# Autodesk Inventor assembly: plate attachment _MIR
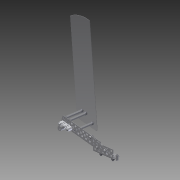
[picture p0: Inventor's stored thumbnail of the model, 180x180]
Saved by Autodesk Inventor 2014 SP1 (Build 180222100, 222)
## iProperties
Created: 2014-03-20
Part Number: plate attachment _MIR
Document SubType Name: Assembly
Designer: Ryan
Author: Ryan
## Documents named in this file (15)
- C:\Users\Ryan\Desktop\sw\toss up 5th A bot\intake\plate attachment _MIR.iam
- C:\Users\Ryan\Desktop\sw\lib\Aperture VEX CAD Library\Metal\L Bar\2 x 5.ipt
- C:\Users\Ryan\Desktop\sw\lib\Aperture VEX CAD Library\Metal\L Bar\2 x 10.ipt
- C:\Users\Ryan\Desktop\sw\lib\Aperture VEX CAD Library\Hardware\8-32\8-32_.375.ipt
- C:\Users\Ryan\Desktop\sw\lib\Aperture VEX CAD Library\Hardware\8-32\8-32 nylock_MIR12.ipt
- C:\Users\Ryan\Desktop\sw\lib\Aperture VEX CAD Library\Metal\Custom 1 bar\5.ipt
- C:\Users\Ryan\Desktop\sw\lib\Aperture VEX CAD Library\Hardware\8-32\8-32 nylock.ipt
- C:\Users\Ryan\Desktop\sw\lib\Aperture VEX CAD Library\Bearing Blocks\Bearing Block.ipt
- C:\Users\Ryan\Desktop\sw\lib\Aperture VEX CAD Library\Hardware\8-32\8-32_.250.ipt
- C:\Users\Ryan\Desktop\sw\lib\Aperture VEX CAD Library\Standoffs\BEAM-0500.ipt
- C:\Users\Ryan\Desktop\sw\lib\Aperture VEX CAD Library\Standoffs\BEAM-2000.ipt
- C:\Users\Ryan\Desktop\sw\lib\Aperture VEX CAD Library\Hardware\8-32\8-23_.750.ipt
- C:\Users\Ryan\Desktop\sw\lib\Aperture VEX CAD Library\Spacers\SPACER-0500-0125.ipt
- C:\Users\Ryan\Desktop\sw\lib\Aperture VEX CAD Library\Spacers\SPACER-0500-0375.ipt
- C:\Users\Ryan\Desktop\sw\toss up 5th A bot\intake\large ball holder.ipt
## Components (36 placed, 14 different names)
1. 2 x 5:1 — Mate:31, Mate:30, Mate:29, Mate:28, Mate:36, Mate:38, Mate:37, Mate:44, Mate:66, Mate:65, Mate:64, Mate:67, Mate:70, Mate:69, Mate:68, Flush:1
2. 2 x 10:1 — Mate:31, Mate:33, Mate:32, Mate:35, Mate:46, Mate:45, Mate:51, Mate:86, Mate:62, Mate:59, Mate:60, Mate:92, Mate:91, Mate:83, Mate:90, Mate:97, Mate:96, Mate:95
3. 8-32_.375:1 — Mate:33, Mate:32, Mate:30, Mate:29, Mate:28, Mate:34
4. 8-32 nylock_MIR12:1 — Mate:35, Mate:34
5. 5:1 — Mate:36, Mate:43, Mate:42, Mate:41, Mate:49, Mate:48, Mate:47
6. 8-32_.375:2 — Mate:43, Mate:42, Mate:41, Mate:38, Mate:37, Mate:40
7. 8-32 nylock:1 — Mate:44, Mate:40
8. 8-32_.375:3 — Mate:49, Mate:48, Mate:47, Mate:46, Mate:45, Mate:50
9. 8-32 nylock:2 — Mate:51, Mate:50
10. Bearing Block:1 — Mate:86, Mate:62, Mate:59, Mate:58, Mate:57, Mate:56, Mate:87
11. Bearing Block:2 — Mate:60, Mate:58, Mate:57, Mate:56, Mate:88, Mate:103, Mate:102
12. 8-32_.250:1 — Mate:70, Mate:69, Mate:68, Mate:71
13. BEAM-0500:1 — Flush:1, Mate:71
14. BEAM-2000:2 — Mate:93, Mate:94, Mate:99, Mate:98
15. 8-32 nylock:6 — Mate:97, Mate:96, Mate:95, Mate:93, Mate:94
16. 8-32 nylock:7 — Mate:99, Mate:98, Mate:107, Mate:106, Mate:66
17. SPACER-0500-0125:1 — Mate:103, Mate:102, Mate:105, Mate:104
18. SPACER-0500-0375:1 — Mate:105, Mate:104
19. 8-32_.375:5 — Mate:107, Mate:106, Mate:69
20. large ball holder:1 — Mate:66, Mate:69, Mate:70
21. 8-32 nylock:3 — Mate:67, Mate:63
22. 8-32_.375:4 — Mate:66, Mate:65, Mate:64, Mate:63
23. 8-32 nylock:9
24. 8-32_.375:7
25. 8-23_.750:1 — Mate:89, Mate:88, Mate:87
26. 8-32 nylock:5 — Mate:90, Mate:89
27. 8-23_.750:2
28. 8-32 nylock:10
29. BEAM-2000:1 — Mate:85, Mate:84, Mate:101, Mate:100
30. 8-32 nylock:4 — Mate:92, Mate:91, Mate:85, Mate:84, Mate:83
31. 8-32 nylock:8 — Mate:101, Mate:100, Mate:109, Mate:108
32. 8-32_.375:6 — Mate:109, Mate:108
33. BEAM-2000:3
34. 8-32 nylock:11
35. 8-32 nylock:12
36. 8-32_.375:8 — Mate:70
## Component patterns: (2 elements, first: 8-32 nylock:3 + 8-32_.375:4), (2 elements, first: 8-23_.750:1 + 8-32 nylock:5), (2 elements, first: BEAM-2000:1 + 8-32 nylock:4 + 8-32 nylock:8 + 8-32_.375:6)
## Relationships (69: Mate 68, Flush 1)
- Mate:31: 2 x 5:1 ↔ 2 x 10:1
- Mate:33 (2.3114 mm): 2 x 10:1 ↔ 8-32_.375:1
- Mate:32 (2.3114 mm): 2 x 10:1 ↔ 8-32_.375:1
- Mate:30 (2.3114 mm): 2 x 5:1 ↔ 8-32_.375:1
- Mate:29 (2.3114 mm): 2 x 5:1 ↔ 8-32_.375:1
- Mate:28: 2 x 5:1 ↔ 8-32_.375:1
- Mate:35: 2 x 10:1 ↔ 8-32 nylock_MIR12:1
- Mate:34: 8-32_.375:1 ↔ 8-32 nylock_MIR12:1
- Mate:36: 2 x 5:1 ↔ 5:1
- Mate:43: 5:1 ↔ 8-32_.375:2
- Mate:42 (2.3114 mm): 5:1 ↔ 8-32_.375:2
- Mate:41 (2.3114 mm): 5:1 ↔ 8-32_.375:2
- Mate:38 (2.3114 mm): 2 x 5:1 ↔ 8-32_.375:2
- Mate:37 (2.3114 mm): 2 x 5:1 ↔ 8-32_.375:2
- Mate:44: 2 x 5:1 ↔ 8-32 nylock:1
- Mate:40: 8-32_.375:2 ↔ 8-32 nylock:1
- Mate:49: 5:1 ↔ 8-32_.375:3
- Mate:48 (2.3114 mm): 5:1 ↔ 8-32_.375:3
- Mate:47 (2.3114 mm): 5:1 ↔ 8-32_.375:3
- Mate:46 (2.3114 mm): 2 x 10:1 ↔ 8-32_.375:3
- Mate:45 (2.3114 mm): 2 x 10:1 ↔ 8-32_.375:3
- Mate:51: 2 x 10:1 ↔ 8-32 nylock:2
- Mate:50: 8-32_.375:3 ↔ 8-32 nylock:2
- Mate:86 (2.3114 mm): 2 x 10:1 ↔ Bearing Block:1
- Mate:62 (27.7114 mm): 2 x 10:1 ↔ Bearing Block:1
- Mate:59: 2 x 10:1 ↔ Bearing Block:1
- Mate:60 (-23.0886 mm): 2 x 10:1 ↔ Bearing Block:2
- Mate:58: Bearing Block:1 ↔ Bearing Block:2
- Mate:57: Bearing Block:1 ↔ Bearing Block:2
- Mate:56: Bearing Block:1 ↔ Bearing Block:2
- Mate:66 (2.3114 mm): 2 x 5:1 ↔ 8-32_.375:4
- Mate:65 (2.3114 mm): 2 x 5:1 ↔ 8-32_.375:4
- Mate:64: 2 x 5:1 ↔ 8-32_.375:4
- Mate:67 (1.1684 mm): 2 x 5:1 ↔ 8-32 nylock:3
- Mate:63: 8-32 nylock:3 ↔ 8-32_.375:4
- Mate:70 (2.3114 mm): 2 x 5:1 ↔ 8-32_.250:1
- Mate:69 (1.1684 mm): 2 x 5:1 ↔ 8-32_.250:1
- Mate:68 (15.0114 mm): 2 x 5:1 ↔ 8-32_.250:1
- Flush:1: 2 x 5:1 ↔ BEAM-0500:1
- Mate:71: 8-32_.250:1 ↔ BEAM-0500:1
- Mate:92 (-23.0886 mm): 2 x 10:1 ↔ 8-32 nylock:4
- Mate:91 (2.3114 mm): 2 x 10:1 ↔ 8-32 nylock:4
- Mate:85: BEAM-2000:1 ↔ 8-32 nylock:4
- Mate:84: BEAM-2000:1 ↔ 8-32 nylock:4
- Mate:83: 2 x 10:1 ↔ 8-32 nylock:4
- Mate:90: 2 x 10:1 ↔ 8-32 nylock:5
- Mate:89: 8-23_.750:1 ↔ 8-32 nylock:5
- Mate:88: Bearing Block:2 ↔ 8-23_.750:1
- Mate:87: Bearing Block:1 ↔ 8-23_.750:1
- Mate:97: 2 x 10:1 ↔ 8-32 nylock:6
- Mate:96 (-23.0886 mm): 2 x 10:1 ↔ 8-32 nylock:6
- Mate:95 (2.3114 mm): 2 x 10:1 ↔ 8-32 nylock:6
- Mate:93: BEAM-2000:2 ↔ 8-32 nylock:6
- Mate:94: BEAM-2000:2 ↔ 8-32 nylock:6
- Mate:99: BEAM-2000:2 ↔ 8-32 nylock:7
- Mate:98: BEAM-2000:2 ↔ 8-32 nylock:7
- Mate:101: BEAM-2000:1 ↔ 8-32 nylock:8
- Mate:100: BEAM-2000:1 ↔ 8-32 nylock:8
- Mate:103: Bearing Block:2 ↔ SPACER-0500-0125:1
- Mate:102: Bearing Block:2 ↔ SPACER-0500-0125:1
- Mate:105: SPACER-0500-0125:1 ↔ SPACER-0500-0375:1
- Mate:104: SPACER-0500-0125:1 ↔ SPACER-0500-0375:1
- Mate:107 (1.5875 mm): 8-32 nylock:7 ↔ 8-32_.375:5
- Mate:106: 8-32 nylock:7 ↔ 8-32_.375:5
- Mate:109 (1.5875 mm): 8-32 nylock:8 ↔ 8-32_.375:6
- Mate:108: 8-32 nylock:8 ↔ 8-32_.375:6
- Mate:66: 8-32 nylock:7 ↔ large ball holder:1
- Mate:69: 8-32_.375:5 ↔ large ball holder:1
- Mate:70: large ball holder:1 ↔ 8-32_.375:8
